# Autodesk Inventor assembly: baseProtoPress
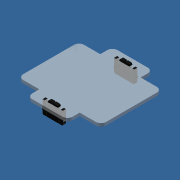
[picture p0: Inventor's stored thumbnail of the model, 180x180]
Saved by Autodesk Inventor 2014 (Build 180170000, 170)
## iProperties
Created: 2014-02-13
Part Number: baseProtoPress
Document SubType Name: Assembly
Designer: Lefo
Author: Lefo
## Documents named in this file (3)
- C:\Users\Lefo\Documents\Inventor\arduinoUno\pressfit\baseProtoPress.iam
- C:\Users\Lefo\Documents\Inventor\arduinoUno\pressfit\base protopress.ipt
- C:\Users\Lefo\Documents\Inventor\arduinoUno\pressfit\pressfit1press.ipt
## Components (3 placed, 2 different names)
1. base protopress:1 — Mate:1, Mate:2, Mate:3, Mate:4, Mate:5, Mate:6
2. pressfit1press:1 — Mate:1, Mate:2, Mate:3
3. pressfit1press:2 — Mate:4, Mate:5, Mate:6
## Relationships (6: Mate 6)
- Mate:1: base protopress:1 ↔ pressfit1press:1
- Mate:2: base protopress:1 ↔ pressfit1press:1
- Mate:3: base protopress:1 ↔ pressfit1press:1
- Mate:4: base protopress:1 ↔ pressfit1press:2
- Mate:5: base protopress:1 ↔ pressfit1press:2
- Mate:6: base protopress:1 ↔ pressfit1press:2
